# Autodesk Inventor assembly: completeAssembly
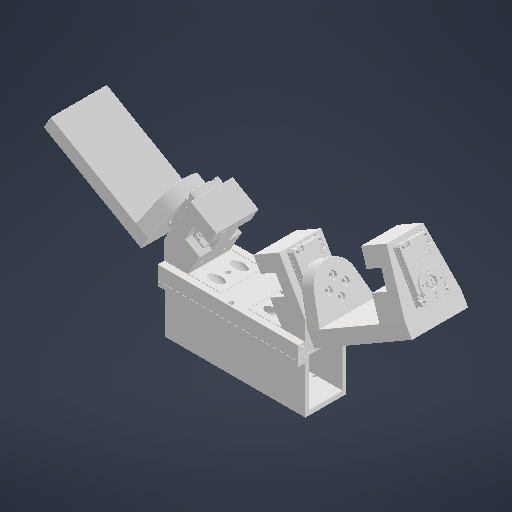
[picture p0: Inventor's stored thumbnail of the model, 512x512]
Saved by Autodesk Inventor 2026 (Build 300175000, 175)
## iProperties
Created: 2025-04-15
Part Number: completeAssembly
Document SubType Name: Assembly
Designer: Elizabeth
Author: Elizabeth
## Documents named in this file (7)
- C:\Users\Elizabeth\FrontierLab\firstMockup\completeAssembly.iam
- C:\Users\Elizabeth\FrontierLab\firstMockup\centralBody.ipt
- C:\Users\Elizabeth\FrontierLab\firstMockup\motorHousing.ipt
- C:\Users\Elizabeth\FrontierLab\firstMockup\controllerHousing.ipt
- C:\Users\Elizabeth\FrontierLab\firstMockup\DYNAMIXEL\DYNAMIXEL_XL330XL,XC-330.iam
- C:\Users\Elizabeth\FrontierLab\firstMockup\rearTorso.ipt
- C:\Users\Elizabeth\FrontierLab\firstMockup\frontTorso.ipt
## Components (9 placed, 6 different names)
1. centralBody:1 — Mate:1, Flush:1, Mate:2, Mate:3, Flush:2, Mate:4, Mate:5, Flush:3, Flush:4, Flush:5, Flush:6
2. motorHousing:1 — Mate:1, Flush:1, Mate:2, Mate:6, Mate:7, Mate:8
3. motorHousing:2 — Mate:3, Flush:2, Mate:4, Mate:9, Mate:10, Mate:11
4. controllerHousing:1 — Mate:5, Flush:3, Flush:4
5. DYNAMIXEL_XL330XL,XC-330:1 [sub-assembly] — Mate:6, Mate:7, Mate:8, Mate:15, Mate:16
6. DYNAMIXEL_XL330XL,XC-330:2 [sub-assembly] — Mate:9, Mate:10, Mate:11, Mate:13, Mate:14
7. rearTorso:1 — Mate:13, Flush:5, Mate:14
8. frontTorso:1 — Mate:15, Mate:16, Flush:6, Mate:17, Mate:18, Mate:19
9. DYNAMIXEL_XL330XL,XC-330:3 [sub-assembly] — Mate:17, Mate:18, Mate:19
## Relationships (24: Mate 18, Flush 6)
- Mate:1 (0.3 mm): centralBody:1 ↔ motorHousing:1
- Flush:1: centralBody:1 ↔ motorHousing:1
- Mate:2 (0.3 mm): centralBody:1 ↔ motorHousing:1
- Mate:3 (0.3 mm): centralBody:1 ↔ motorHousing:2
- Flush:2: centralBody:1 ↔ motorHousing:2
- Mate:4 (0.3 mm): centralBody:1 ↔ motorHousing:2
- Mate:5: centralBody:1 ↔ controllerHousing:1
- Flush:3: centralBody:1 ↔ controllerHousing:1
- Flush:4: centralBody:1 ↔ controllerHousing:1
- Mate:6 (0.1 mm): motorHousing:1 ↔ DYNAMIXEL_XL330XL,XC-330:1
- Mate:7 (0.1 mm): motorHousing:1 ↔ DYNAMIXEL_XL330XL,XC-330:1
- Mate:8 (0.1 mm): motorHousing:1 ↔ DYNAMIXEL_XL330XL,XC-330:1
- Mate:9 (0.1 mm): motorHousing:2 ↔ DYNAMIXEL_XL330XL,XC-330:2
- Mate:10 (0.1 mm): motorHousing:2 ↔ DYNAMIXEL_XL330XL,XC-330:2
- Mate:11 (0.1 mm): motorHousing:2 ↔ DYNAMIXEL_XL330XL,XC-330:2
- Mate:13: DYNAMIXEL_XL330XL,XC-330:2 ↔ rearTorso:1
- Flush:5: centralBody:1 ↔ rearTorso:1
- Mate:14 (0.3 mm): DYNAMIXEL_XL330XL,XC-330:2 ↔ rearTorso:1
- Mate:15: DYNAMIXEL_XL330XL,XC-330:1 ↔ frontTorso:1
- Mate:16 (0.3 mm): DYNAMIXEL_XL330XL,XC-330:1 ↔ frontTorso:1
- Flush:6: centralBody:1 ↔ frontTorso:1
- Mate:17 (0.1 mm): frontTorso:1 ↔ DYNAMIXEL_XL330XL,XC-330:3
- Mate:18 (0.1 mm): frontTorso:1 ↔ DYNAMIXEL_XL330XL,XC-330:3
- Mate:19 (0.1 mm): frontTorso:1 ↔ DYNAMIXEL_XL330XL,XC-330:3
